# Autodesk Inventor assembly: Camera-case
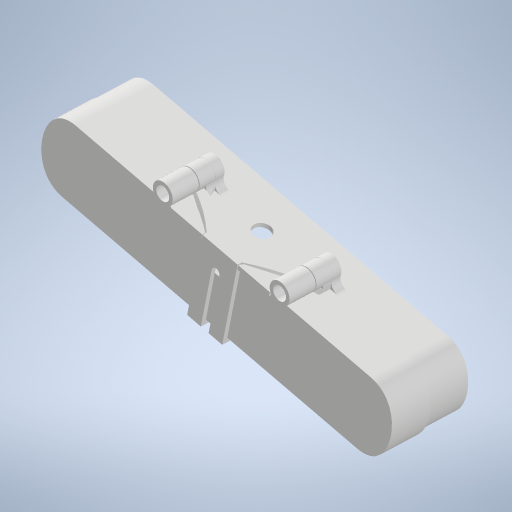
[picture p0: Inventor's stored thumbnail of the model, 512x512]
Saved by Autodesk Inventor 2023 (Build 270158000, 158)
## iProperties
Created: 2022-12-02
Part Number: Camera-case
Document SubType Name: Assembly
Designer: t205b
Author: t205b
## Documents named in this file (4)
- C:\Users\t205b\OneDrive\Documents\PSU Extracuriculars\Robotics\URC Camera\CO-0-01-cameraCase.iam
- C:\Users\t205b\OneDrive\Documents\PSU Extracuriculars\Robotics\URC Camera\CO-1-01-cameraFront.ipt
- C:\Users\t205b\OneDrive\Documents\PSU Extracuriculars\Robotics\URC Camera\CO-1-01-cameraBack.ipt
- C:\Users\t205b\OneDrive\Documents\PSU Extracuriculars\Robotics\URC Camera\CO-1-01-cameraConnector.ipt
## Components (3 placed, 3 different names)
1. CO-1-01-cameraFront:1 — Mate:1, Flush:1, Mate:2, Mate:3
2. CO-1-01-cameraBack:1 — Mate:1, Flush:1, Mate:2, Mate:4, Mate:5
3. CO-1-01-cameraConnector:1 — Mate:3, Mate:4, Mate:5
## Relationships (6: Mate 5, Flush 1)
- Mate:1: CO-1-01-cameraFront:1 ↔ CO-1-01-cameraBack:1
- Flush:1: CO-1-01-cameraFront:1 ↔ CO-1-01-cameraBack:1
- Mate:2: CO-1-01-cameraFront:1 ↔ CO-1-01-cameraBack:1
- Mate:3: CO-1-01-cameraFront:1 ↔ CO-1-01-cameraConnector:1
- Mate:4: CO-1-01-cameraBack:1 ↔ CO-1-01-cameraConnector:1
- Mate:5: CO-1-01-cameraBack:1 ↔ CO-1-01-cameraConnector:1
